# Autodesk Inventor assembly: PCB enclosure
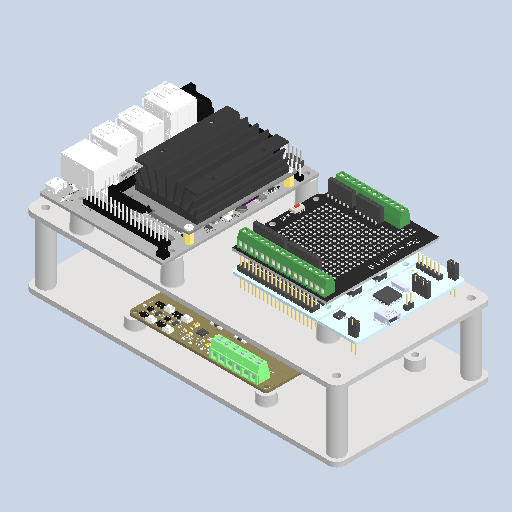
[picture p0: Inventor's stored thumbnail of the model, 512x512]
Saved by Autodesk Inventor 2026 (Build 300175050, 175E)
## iProperties
Created: 2025-10-28
Part Number: PCB enclosure
Document SubType Name: Assembly
Designer: Kartik
Mass: 248.178 g
Surface Area: 2728.95 cm^2
Volume: 248.178 cm^3
Density: 1 g/cm^3
Author: Kartik
## Documents named in this file (8)
- D:\Kartik\Projects\AMR\CAD\2 Sub-assembly\PCB enclosure.iam
- D:\Kartik\Projects\AMR\CAD\4 Boughtouts\MDD20A CAD\MDD20A\MDD20A\MDD20A.ipt
- D:\Kartik\Projects\AMR\CAD\4 Boughtouts\NUCLEO-F401RE--3DModel-STEP-56544\NUCLEO-F401RE--3DModel-STEP-56544\NUCLEO-F401RE--3DModel-STEP-56544.ipt
- D:\Kartik\Projects\AMR\CAD\4 Boughtouts\nvidia-jetson-nano-4gb\Jetson nano 4GB\Jetson nano 4GB\Jetson nano 4GB.ipt
- D:\Kartik\Projects\AMR\CAD\3 Parts\Base_MDD20A.ipt
- D:\Kartik\Projects\AMR\CAD\3 Parts\Base_ST_nano.ipt
- D:\Kartik\Projects\AMR\CAD\3 Parts\Spacer.ipt
- D:\Kartik\Projects\AMR\CAD\4 Boughtouts\arduino-uno-screw-shield-1\Arduino Uno Screw Shield\Arduino Uno Screw Shield\Arduino Uno Screw Shield.ipt
## Components (10 placed, 7 different names)
1. MDD20A:1 — Mate:1, Flush:8, Mate:7, Mate:8, Mate:9, Angle:2
2. NUCLEO-F401RE--3DModel-STEP-56544:1 — Mate:1, Flush:9, Flush:8, Mate:6, Mate:17, Mate:18, Mate:25, Mate:26, Mate:27
3. Jetson nano 4GB:1 — Flush:9, Angle:1, Mate:11, Mate:15, Mate:16
4. Base_MDD20A:1 — Mate:7, Mate:8, Mate:9, Angle:2, Flush:10, Mate:19, Mate:20, Mate:21, Mate:22, Mate:23, Mate:24
5. Base_ST_nano:1 — Mate:11, Flush:10, Mate:15, Mate:16, Mate:17, Mate:18
6. Spacer:1 — Mate:19, Mate:20
7. Spacer:2 — Flush:11, Mate:24
8. Spacer:3 — Flush:11, Flush:12, Mate:23
9. Spacer:4 — Flush:12, Mate:21, Mate:22
10. Arduino Uno Screw Shield:1 — Mate:25, Mate:26, Mate:27
## Relationships (26: Mate 19, Flush 5, Angle 2)
- Mate:1 (50 mm): MDD20A:1 ↔ NUCLEO-F401RE--3DModel-STEP-56544:1
- Flush:9: NUCLEO-F401RE--3DModel-STEP-56544:1 ↔ Jetson nano 4GB:1
- Flush:8: MDD20A:1 ↔ NUCLEO-F401RE--3DModel-STEP-56544:1
- Angle:1 (0 deg): Jetson nano 4GB:1
- Mate:6: NUCLEO-F401RE--3DModel-STEP-56544:1
- Mate:7: MDD20A:1 ↔ Base_MDD20A:1
- Mate:8 (-2.5 mm): MDD20A:1 ↔ Base_MDD20A:1
- Mate:9 (-2.5 mm): MDD20A:1 ↔ Base_MDD20A:1
- Angle:2 (0 deg): MDD20A:1 ↔ Base_MDD20A:1
- Mate:11: Jetson nano 4GB:1 ↔ Base_ST_nano:1
- Flush:10: Base_MDD20A:1 ↔ Base_ST_nano:1
- Mate:15: Jetson nano 4GB:1 ↔ Base_ST_nano:1
- Mate:16: Jetson nano 4GB:1 ↔ Base_ST_nano:1
- Mate:17: NUCLEO-F401RE--3DModel-STEP-56544:1 ↔ Base_ST_nano:1
- Mate:18: NUCLEO-F401RE--3DModel-STEP-56544:1 ↔ Base_ST_nano:1
- Mate:19: Base_MDD20A:1 ↔ Spacer:1
- Mate:20: Base_MDD20A:1 ↔ Spacer:1
- Flush:11: Spacer:2 ↔ Spacer:3
- Flush:12: Spacer:3 ↔ Spacer:4
- Mate:21: Base_MDD20A:1 ↔ Spacer:4
- Mate:22: Base_MDD20A:1 ↔ Spacer:4
- Mate:23: Base_MDD20A:1 ↔ Spacer:3
- Mate:24: Base_MDD20A:1 ↔ Spacer:2
- Mate:25: NUCLEO-F401RE--3DModel-STEP-56544:1 ↔ Arduino Uno Screw Shield:1
- Mate:26: NUCLEO-F401RE--3DModel-STEP-56544:1 ↔ Arduino Uno Screw Shield:1
- Mate:27: NUCLEO-F401RE--3DModel-STEP-56544:1 ↔ Arduino Uno Screw Shield:1
